# Autodesk Inventor assembly: v6
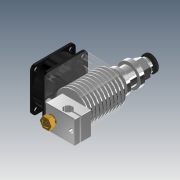
[picture p0: Inventor's stored thumbnail of the model, 180x180]
Saved by Autodesk Inventor 2021 (Build 250183000, 183)
## iProperties
Created: 2023-03-21
Part Number: v6
Document SubType Name: Assembly
Designer: WubbGmbaa
Author: WubbGmbaa
## Documents named in this file (8)
- G:\Misc\makerspace\TAZ\hybrid-hotend-refactor\ref\v6.iam
- G:\Misc\makerspace\TAZ\hybrid-hotend-refactor\ref\e3d\v6-hotend-heatsink.ipt
- G:\Misc\makerspace\TAZ\hybrid-hotend-refactor\ref\e3d\fan.ipt
- G:\Misc\makerspace\TAZ\hybrid-hotend-refactor\ref\e3d\bowden-adapter-coldend.ipt
- G:\Misc\makerspace\TAZ\hybrid-hotend-refactor\ref\e3d\e3d heat break.ipt
- G:\Misc\makerspace\TAZ\hybrid-hotend-refactor\ref\e3d\e3d heaterblock.ipt
- G:\Misc\makerspace\TAZ\hybrid-hotend-refactor\ref\e3d\e3d nozzle (0.4).ipt
- G:\Misc\makerspace\TAZ\hybrid-hotend-refactor\ref\e3d\fan duct.ipt
## Components (7 placed, 7 different names)
1. v6-hotend-heatsink:1 — Insert:1, Insert:2, Mate:1, Flush:2
2. bowden-adapter-coldend:1 — Insert:1
3. e3d heat break:1 — Insert:2, Insert:3
4. e3d heaterblock:1 — Insert:3, Insert:4, Angle:1
5. e3d nozzle (0.4):1 — Insert:4
6. fan duct:1 — Mate:1, Flush:1, Angle:1, Insert:5
7. fan:1 — Insert:5
## Relationships (9: Insert 5, Flush 2, Mate 1, Angle 1)
- Insert:1: v6-hotend-heatsink:1 ↔ bowden-adapter-coldend:1
- Insert:2: v6-hotend-heatsink:1 ↔ e3d heat break:1
- Insert:3: e3d heat break:1 ↔ e3d heaterblock:1
- Insert:4: e3d heaterblock:1 ↔ e3d nozzle (0.4):1
- Mate:1: v6-hotend-heatsink:1 ↔ fan duct:1
- Flush:1: fan duct:1
- Flush:2: v6-hotend-heatsink:1
- Angle:1 (0 deg): e3d heaterblock:1 ↔ fan duct:1
- Insert:5: fan duct:1 ↔ fan:1
